# Autodesk Inventor assembly: ARM_031_TwoPieceIntake
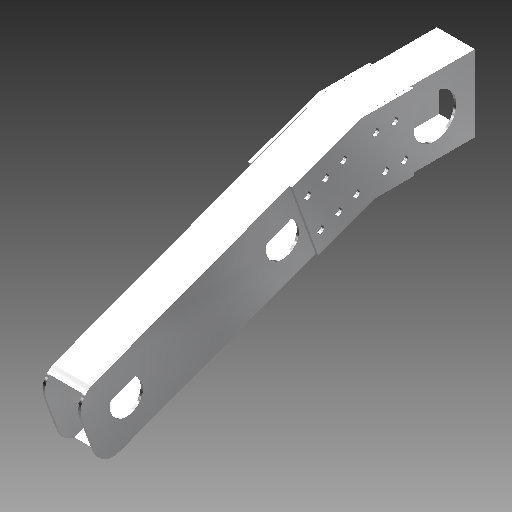
[picture p0: Inventor's stored thumbnail of the model, 512x512]
Saved by Autodesk Inventor 2018.3 (Build 223284000, 284)
## iProperties
Created: 2020-02-04
Part Number: ARM_031_TwoPieceIntake
Document SubType Name: Assembly
Designer: 22turnmaxw
Mass: 158.095 g
Surface Area: 753.685 cm^2
Volume: 58.5538 cm^3
Density: 2.7 g/cm^3
Author: 22turnmaxw
## Documents named in this file (4)
- C:\Users\22oktynich\Documents\GrabCAD\Infinite Recharge 2020\Build season\ARM_031_TwoPieceIntake.iam
- C:\Users\22oktynich\Documents\GrabCAD\Infinite Recharge 2020\Build season\ARM_029_BottomIntakeSide.ipt
- C:\Users\22oktynich\Documents\GrabCAD\Infinite Recharge 2020\Build season\ARM_030_TopIntakeSide.ipt
- C:\Users\22oktynich\Documents\GrabCAD\Infinite Recharge 2020\Build season\ARM_073_TwoPieceIntakeGusset.ipt
## Components (4 placed, 3 different names)
1. ARM_029_BottomIntakeSide:1 — Mate:2, Mate:3, Mate:4, Mate:5, Flush:1, Mate:6, Mate:7, Flush:2, Mate:8
2. ARM_030_TopIntakeSide:1 — Mate:2, Mate:3, Mate:4
3. ARM_073_TwoPieceIntakeGusset:1 — Mate:5, Flush:1, Mate:6
4. ARM_073_TwoPieceIntakeGusset:2 — Mate:7, Flush:2, Mate:8
## Relationships (9: Mate 7, Flush 2)
- Mate:2 (-25.4 mm): ARM_029_BottomIntakeSide:1 ↔ ARM_030_TopIntakeSide:1
- Mate:3: ARM_029_BottomIntakeSide:1 ↔ ARM_030_TopIntakeSide:1
- Mate:4: ARM_029_BottomIntakeSide:1 ↔ ARM_030_TopIntakeSide:1
- Mate:5: ARM_029_BottomIntakeSide:1 ↔ ARM_073_TwoPieceIntakeGusset:1
- Flush:1: ARM_029_BottomIntakeSide:1 ↔ ARM_073_TwoPieceIntakeGusset:1
- Mate:6: ARM_029_BottomIntakeSide:1 ↔ ARM_073_TwoPieceIntakeGusset:1
- Mate:7: ARM_029_BottomIntakeSide:1 ↔ ARM_073_TwoPieceIntakeGusset:2
- Flush:2: ARM_029_BottomIntakeSide:1 ↔ ARM_073_TwoPieceIntakeGusset:2
- Mate:8: ARM_029_BottomIntakeSide:1 ↔ ARM_073_TwoPieceIntakeGusset:2
